# Autodesk Inventor assembly: wheel-assembly
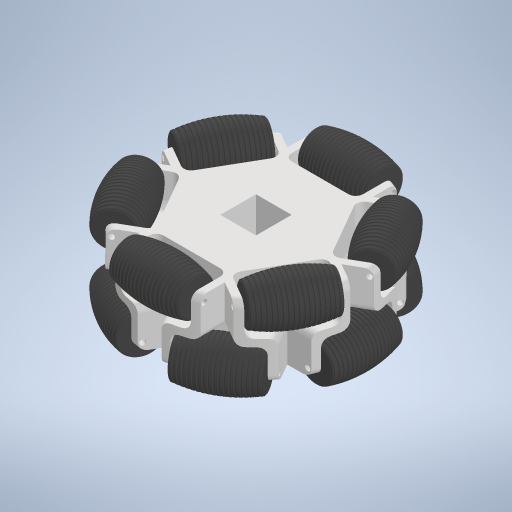
[picture p0: Inventor's stored thumbnail of the model, 512x512]
Saved by Autodesk Inventor 2024.2 (Build 282272000, 272)
## iProperties
Created: 2024-04-23
Part Number: wheel-assembly
Document SubType Name: Assembly
Designer: Robin
Author: Robin
## Documents named in this file (3)
- C:\Users\Robin\OneDrive\Study\Current\Mechanical Design\Cad\fork-cad\wheel-assembly.iam
- C:\Users\Robin\OneDrive\Study\Current\Mechanical Design\Cad\fork-cad\holo-6-wheel.ipt
- C:\Users\Robin\OneDrive\Study\Current\Mechanical Design\Cad\fork-cad\roller-6.ipt
## Components (13 placed, 2 different names)
1. holo-6-wheel:1 — Mate:1, Mate:2, Mate:3, Mate:4
2. roller-6:1 — Mate:1, Mate:2
3. roller-6:2
4. roller-6:3
5. roller-6:4
6. roller-6:5
7. roller-6:6
8. roller-6:7 — Mate:3, Mate:4
9. roller-6:8
10. roller-6:9
11. roller-6:10
12. roller-6:11
13. roller-6:12
## Component patterns: (6 elements, first: roller-6:1), (6 elements, first: roller-6:7)
## Relationships (4: Mate 4)
- Mate:1: holo-6-wheel:1 ↔ roller-6:1
- Mate:2 (0.25 mm): holo-6-wheel:1 ↔ roller-6:1
- Mate:3 (0.25 mm): holo-6-wheel:1 ↔ roller-6:7
- Mate:4: holo-6-wheel:1 ↔ roller-6:7
